# Autodesk Inventor assembly: FullBuild
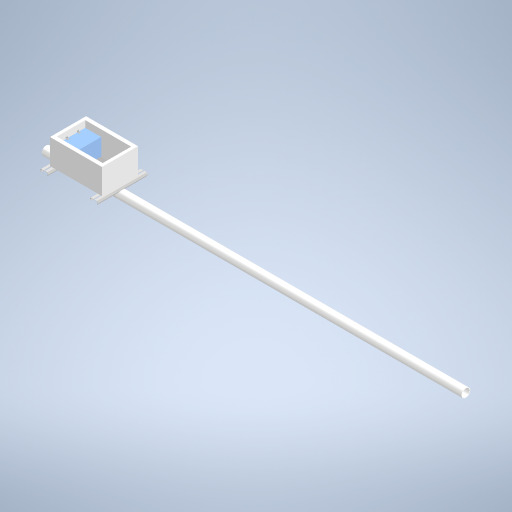
[picture p0: Inventor's stored thumbnail of the model, 512x512]
Saved by Autodesk Inventor 2024.2 (Build 282272000, 272)
## iProperties
Created: 2024-01-15
Part Number: FullBuild
Document SubType Name: Assembly
Designer: airso
Author: airso
## Documents named in this file (9)
- C:\Users\airso\OneDrive\Documents\school\2023 Fall\Capstone\Inventor Files\FullBuild.iam
- C:\Users\airso\OneDrive\Documents\school\2023 Fall\Capstone\Inventor Files\2x8PVC.ipt
- C:\Users\airso\OneDrive\Documents\school\2023 Fall\Capstone\Inventor Files\JunctionBox.ipt
- C:\Users\airso\OneDrive\Documents\school\2023 Fall\Capstone\Inventor Files\PoleBracket.ipt
- C:\Users\airso\OneDrive\Documents\school\2023 Fall\Capstone\Inventor Files\PoleWrap.ipt
- C:\Users\airso\OneDrive\Documents\school\2023 Fall\Capstone\Inventor Files\97763A213_18-8 Stainless Steel Button Head Hex Drive Screws\97763A213_18-8 Stainless Steel Button Head Hex Drive Screws.ipt
- C:\Users\airso\OneDrive\Documents\school\2023 Fall\Capstone\Inventor Files\Cablepipe.ipt
- C:\Users\airso\OneDrive\Documents\school\2023 Fall\Capstone\Inventor Files\1959N41_Corner Bracket for Single Rail Miniature T-Slotted Framing\1959N41_Corner Bracket for Single Rail Miniature T-Slotted Framing.ipt
- C:\Users\airso\OneDrive\Documents\school\2023 Fall\Capstone\Inventor Files\99461A171_Phillips Rounded Head Thread-Forming Screws\99461A171_Phillips Rounded Head Thread-Forming Screws.ipt
## Components (19 placed, 8 different names)
1. 2x8PVC:1 — Mate:13, Flush:3
2. JunctionBox:1 — Mate:1, Mate:2, Mate:3, Mate:4, Mate:5, Mate:6, Flush:1, Flush:2, Mate:8, Mate:9, Mate:11, Mate:12, Flush:3, Mate:14, Mate:17, Mate:19, Mate:21, Mate:22, Mate:23, Mate:24, Mate:25, Mate:26, Mate:27, Mate:28, Mate:29, Mate:34, Mate:35, Mate:36, Mate:37, Mate:38, Mate:39, Mate:40, Mate:41
3. PoleBracket:1 — Mate:2, Mate:3, Mate:4, Flush:1, Mate:7, Mate:15, Mate:16
4. PoleWrap:1 — Mate:10, Mate:11, Mate:12
5. PoleBracket:2 — Mate:1, Mate:5, Mate:6, Flush:2, Mate:10, Mate:18, Mate:20
6. PoleWrap:2 — Mate:7, Mate:8, Mate:9, Mate:13
7. 97763A213_18-8 Stainless Steel Button Head Hex Drive Screws:1 — Mate:14, Mate:15
8. 97763A213_18-8 Stainless Steel Button Head Hex Drive Screws:2 — Mate:20, Mate:21
9. 97763A213_18-8 Stainless Steel Button Head Hex Drive Screws:3 — Mate:16, Mate:17
10. 97763A213_18-8 Stainless Steel Button Head Hex Drive Screws:4 — Mate:18, Mate:19
11. Cablepipe:1 — Mate:22, Mate:23
12. 1959N41_Corner Bracket for Single Rail Miniature T-Slotted Framing:1 — Mate:24, Mate:26, Mate:28, Mate:30, Mate:31
13. 1959N41_Corner Bracket for Single Rail Miniature T-Slotted Framing:2 — Mate:25, Mate:27, Mate:29, Mate:32, Mate:33
14. 99461A171_Phillips Rounded Head Thread-Forming Screws:1 — Mate:30, Mate:31
15. 99461A171_Phillips Rounded Head Thread-Forming Screws:2 — Mate:32, Mate:33
16. 99461A171_Phillips Rounded Head Thread-Forming Screws:3 — Mate:34, Mate:38
17. 99461A171_Phillips Rounded Head Thread-Forming Screws:4 — Mate:35, Mate:41
18. 99461A171_Phillips Rounded Head Thread-Forming Screws:5 — Mate:36, Mate:40
19. 99461A171_Phillips Rounded Head Thread-Forming Screws:6 — Mate:37, Mate:39
## Relationships (44: Mate 41, Flush 3)
- Mate:1: JunctionBox:1 ↔ PoleBracket:2
- Mate:2: JunctionBox:1 ↔ PoleBracket:1
- Mate:3 (3.556 mm): JunctionBox:1 ↔ PoleBracket:1
- Mate:4 (3.556 mm): JunctionBox:1 ↔ PoleBracket:1
- Mate:5 (3.556 mm): JunctionBox:1 ↔ PoleBracket:2
- Mate:6 (3.556 mm): JunctionBox:1 ↔ PoleBracket:2
- Flush:1 (-40.259 mm): JunctionBox:1 ↔ PoleBracket:1
- Flush:2 (-40.259 mm): JunctionBox:1 ↔ PoleBracket:2
- Mate:7 (36.195 mm): PoleBracket:1 ↔ PoleWrap:2
- Mate:8 (-6.35 mm): JunctionBox:1 ↔ PoleWrap:2
- Mate:9 (-104.775 mm): JunctionBox:1 ↔ PoleWrap:2
- Mate:10 (36.195 mm): PoleWrap:1 ↔ PoleBracket:2
- Mate:11 (-6.35 mm): JunctionBox:1 ↔ PoleWrap:1
- Mate:12 (-104.775 mm): JunctionBox:1 ↔ PoleWrap:1
- Mate:13: 2x8PVC:1 ↔ PoleWrap:2
- Flush:3 (127 mm): 2x8PVC:1 ↔ JunctionBox:1
- Mate:14: JunctionBox:1 ↔ 97763A213_18-8 Stainless Steel Button Head Hex Drive Screws:1
- Mate:15: PoleBracket:1 ↔ 97763A213_18-8 Stainless Steel Button Head Hex Drive Screws:1
- Mate:16: PoleBracket:1 ↔ 97763A213_18-8 Stainless Steel Button Head Hex Drive Screws:3
- Mate:17: JunctionBox:1 ↔ 97763A213_18-8 Stainless Steel Button Head Hex Drive Screws:3
- Mate:18: PoleBracket:2 ↔ 97763A213_18-8 Stainless Steel Button Head Hex Drive Screws:4
- Mate:19: JunctionBox:1 ↔ 97763A213_18-8 Stainless Steel Button Head Hex Drive Screws:4
- Mate:20: PoleBracket:2 ↔ 97763A213_18-8 Stainless Steel Button Head Hex Drive Screws:2
- Mate:21: JunctionBox:1 ↔ 97763A213_18-8 Stainless Steel Button Head Hex Drive Screws:2
- Mate:22: JunctionBox:1 ↔ Cablepipe:1
- Mate:23: JunctionBox:1 ↔ Cablepipe:1
- Mate:24: JunctionBox:1 ↔ 1959N41_Corner Bracket for Single Rail Miniature T-Slotted Framing:1
- Mate:25: JunctionBox:1 ↔ 1959N41_Corner Bracket for Single Rail Miniature T-Slotted Framing:2
- Mate:26: JunctionBox:1 ↔ 1959N41_Corner Bracket for Single Rail Miniature T-Slotted Framing:1
- Mate:27: JunctionBox:1 ↔ 1959N41_Corner Bracket for Single Rail Miniature T-Slotted Framing:2
- Mate:28 (38.1 mm): JunctionBox:1 ↔ 1959N41_Corner Bracket for Single Rail Miniature T-Slotted Framing:1
- Mate:29 (38.1 mm): JunctionBox:1 ↔ 1959N41_Corner Bracket for Single Rail Miniature T-Slotted Framing:2
- Mate:30: 1959N41_Corner Bracket for Single Rail Miniature T-Slotted Framing:1 ↔ 99461A171_Phillips Rounded Head Thread-Forming Screws:1
- Mate:31: 1959N41_Corner Bracket for Single Rail Miniature T-Slotted Framing:1 ↔ 99461A171_Phillips Rounded Head Thread-Forming Screws:1
- Mate:32: 1959N41_Corner Bracket for Single Rail Miniature T-Slotted Framing:2 ↔ 99461A171_Phillips Rounded Head Thread-Forming Screws:2
- Mate:33: 1959N41_Corner Bracket for Single Rail Miniature T-Slotted Framing:2 ↔ 99461A171_Phillips Rounded Head Thread-Forming Screws:2
- Mate:34: JunctionBox:1 ↔ 99461A171_Phillips Rounded Head Thread-Forming Screws:3
- Mate:35: JunctionBox:1 ↔ 99461A171_Phillips Rounded Head Thread-Forming Screws:4
- Mate:36: JunctionBox:1 ↔ 99461A171_Phillips Rounded Head Thread-Forming Screws:5
- Mate:37: JunctionBox:1 ↔ 99461A171_Phillips Rounded Head Thread-Forming Screws:6
- Mate:38: JunctionBox:1 ↔ 99461A171_Phillips Rounded Head Thread-Forming Screws:3
- Mate:39: JunctionBox:1 ↔ 99461A171_Phillips Rounded Head Thread-Forming Screws:6
- Mate:40: JunctionBox:1 ↔ 99461A171_Phillips Rounded Head Thread-Forming Screws:5
- Mate:41: JunctionBox:1 ↔ 99461A171_Phillips Rounded Head Thread-Forming Screws:4
